# Autodesk Inventor assembly: BaseFrame
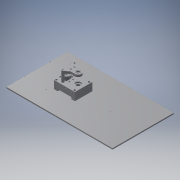
[picture p0: Inventor's stored thumbnail of the model, 180x180]
Saved by Autodesk Inventor 2019 (Build 230136000, 136)
## iProperties
Created: 2020-02-16
Part Number: BaseFrame
Document SubType Name: Assembly
Designer: Alex
Author: Alex
## Documents named in this file (7)
- D:\Alex\Documents\GitHub\RBE3001-URDF-Example\CAD\Inventor_Assembly\Link0.iam
- D:\Alex\Documents\Personal Projects\BenchPowerSupply\basePlateEtching_SVG_Body_part_2.ipt
- D:\Alex\Documents\Personal Projects\BenchPowerSupply\basePlateCut_SVG_Body_part_3.ipt
- D:\Alex\Documents\Personal Projects\BenchPowerSupply\baseRight_Body_part_1.ipt
- D:\Alex\Documents\Personal Projects\BenchPowerSupply\baseLeft_Body_part_0.ipt
- D:\Alex\Documents\Personal Projects\BenchPowerSupply\baseCap_Body_part_4.ipt
- D:\Alex\Documents\GitHub\RBE3001-URDF-Example\CAD\Inventor_Assembly\DriveGear.ipt
## Components (6 placed, 6 different names)
1. basePlateEtching_SVG_Body_part_2:1 — Flush:1, Flush:2, Flush:3
2. basePlateCut_SVG_Body_part_3:1 — Flush:4, Flush:5, Flush:6
3. baseRight_Body_part_1:1 — Flush:7, Flush:8, Flush:9
4. baseLeft_Body_part_0:1 — Flush:10, Flush:11, Flush:12, Mate:1
5. baseCap_Body_part_4:1 — Flush:13, Flush:14, Flush:15
6. DriveGear:1 — Mate:1, Mate:2, Mate:3
## Relationships (18: Flush 15, Mate 3)
- Flush:1: basePlateEtching_SVG_Body_part_2:1
- Flush:2: basePlateEtching_SVG_Body_part_2:1
- Flush:3: basePlateEtching_SVG_Body_part_2:1
- Flush:4: basePlateCut_SVG_Body_part_3:1
- Flush:5: basePlateCut_SVG_Body_part_3:1
- Flush:6: basePlateCut_SVG_Body_part_3:1
- Flush:7: baseRight_Body_part_1:1
- Flush:8: baseRight_Body_part_1:1
- Flush:9: baseRight_Body_part_1:1
- Flush:10: baseLeft_Body_part_0:1
- Flush:11: baseLeft_Body_part_0:1
- Flush:12: baseLeft_Body_part_0:1
- Flush:13: baseCap_Body_part_4:1
- Flush:14: baseCap_Body_part_4:1
- Flush:15: baseCap_Body_part_4:1
- Mate:1: baseLeft_Body_part_0:1 ↔ DriveGear:1
- Mate:2: DriveGear:1
- Mate:3 (-63.75 mm): DriveGear:1
